# Autodesk Inventor assembly: Assembly2タミヤダンパー　上
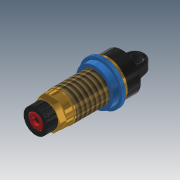
[picture p0: Inventor's stored thumbnail of the model, 180x180]
Saved by Autodesk Inventor 2020.1 (Build 241239000, 239)
## iProperties
Created: 2018-09-18
Part Number: Assembly2タミヤダンパー　上
Material: 一般
Document SubType Name: Assembly
Designer: 杉本　賢二郎
Author: 杉本　賢二郎
## Documents named in this file (7)
- C:\Users\杉本　賢二郎\Desktop\インベンター\新機体制作2020\ダンパー\Assembly2タミヤダンパー_フロント上.iam
- C:\Users\杉本　賢二郎\Desktop\インベンター\新機体制作2020\ダンパー\タミヤダンパー部品1.ipt
- C:\Users\杉本　賢二郎\Desktop\インベンター\新機体制作2020\ダンパー\タミヤダンパー部品3.ipt
- C:\Users\杉本　賢二郎\Desktop\インベンター\新機体制作2020\ダンパー\タミヤダンパー部品4.ipt
- C:\Users\杉本　賢二郎\Desktop\インベンター\新機体制作2020\ダンパー\タミヤダンパー部品8.ipt
- C:\Users\杉本　賢二郎\Desktop\インベンター\新機体制作2020\ダンパー\タミヤダンパー部品6.ipt
- C:\Users\杉本　賢二郎\Desktop\インベンター\新機体制作2020\ダンパー\タミヤダンパー部品2_フロント.ipt
## Components (6 placed, 6 different names)
1. タミヤダンパー部品1:1 — 挿入:4, 挿入:5
2. タミヤダンパー部品3:1 — 挿入:3, 挿入:7
3. タミヤダンパー部品4:1 — 挿入:6
4. タミヤダンパー部品8:1 — 挿入:4
5. タミヤダンパー部品6:1 — 挿入:3
6. タミヤダンパー部品2_フロント:1 — 挿入:5, 挿入:6, 挿入:7
## Relationships (5: Insert 5)
- 挿入:3 [Insert]: タミヤダンパー部品3:1 ↔ タミヤダンパー部品6:1
- 挿入:4 [Insert]: タミヤダンパー部品1:1 ↔ タミヤダンパー部品8:1
- 挿入:5 [Insert]: タミヤダンパー部品1:1 ↔ タミヤダンパー部品2_フロント:1
- 挿入:6 [Insert]: タミヤダンパー部品4:1 ↔ タミヤダンパー部品2_フロント:1
- 挿入:7 [Insert]: タミヤダンパー部品3:1 ↔ タミヤダンパー部品2_フロント:1
